# Autodesk Inventor assembly: Leg V4
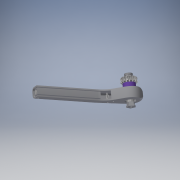
[picture p0: Inventor's stored thumbnail of the model, 180x180]
Saved by Autodesk Inventor 2019.1 (Build 231200000, 200)
## iProperties
Created: 2018-11-28
Part Number: Leg V4
Material: Generisch
Document SubType Name: Assembly
Designer: JochenAlt
Author: JochenAlt
## Documents named in this file (11)
- D:\Projects\Ondine\CAD\Leg\Leg V4.iam
- D:\Projects\Ondine\CAD\Leg\Leg V4.ipt
- D:\Projects\Ondine\CAD\Leg\Leg Inner V4.ipt
- D:\Projects\Ondine\CAD\Leg\LegInnerGear\Synchrone Riemenscheibe21.ipt
- D:\Projects\Ondine\CAD\Leg\LegInnerGear\Synchrone Riemenscheibe11.ipt
- D:\Projects\Ondine\CAD\Leg\LegInnerGear\Flache Riemenscheibe11.ipt
- D:\Projects\Ondine\CAD\Leg\LegInnerGear\Synchrone Riemenscheibe31.ipt
- D:\Projects\Ondine\CAD\Leg\Schnecke\Schneckenrad1.ipt
- D:\Projects\Ondine\CAD\Leg\LegInnerGear\gearNotch.ipt
- D:\Projects\Ondine\CAD\Bearings\W 627_7-2ZS.iam
- D:\Projects\Ondine\CAD\Bearings\W 61700 X-2RS1.iam
## Components (10 placed, 9 different names)
1. Leg:1 — Passend:7, Passend:8, Passend:23, Passend:24, Passend:26, Passend:27, Passend:28, Passend:29, Passend:30, Winkel:3, Passend:40, Passend:42
2. Leg:2 — Passend:41, Passend:42
3. Synchrone Riemenscheibe2:1 — Passend:26, Passend:27, Drehung:2, Passend:41
4. Synchrone Riemenscheibe1:1 — Passend:7, Passend:8, Passend:30
5. Flache Riemenscheibe1:1 — Passend:28, Passend:29
6. Synchrone Riemenscheibe3:1 — Winkel:2, Passend:21, Passend:23, Passend:24, Passend:25, Passend:33, Passend:34
7. LegGearWormPinion:1 — Passend:37, Passend:38, Winkel:3, Passend:39, Passend:40
8. gearNotch:1 — Winkel:2, Passend:21, Passend:25, Drehung:2
9. W 627_7-2ZS:1 [sub-assembly] — Passend:37, Passend:38
10. W 61700 X-2RS1:1 [sub-assembly] — Passend:33, Passend:34, Passend:39
## Relationships (22: Mate 19, Angle 2, RelateRotation 1)
- Passend:7 [Mate]: Leg:1 ↔ Synchrone Riemenscheibe1:1
- Passend:8 [Mate]: Leg:1 ↔ Synchrone Riemenscheibe1:1
- Winkel:2 [Angle] (180 deg): Synchrone Riemenscheibe3:1 ↔ gearNotch:1
- Passend:21 [Mate]: Synchrone Riemenscheibe3:1 ↔ gearNotch:1
- Passend:23 [Mate]: Leg:1 ↔ Synchrone Riemenscheibe3:1
- Passend:24 [Mate]: Leg:1 ↔ Synchrone Riemenscheibe3:1
- Passend:25 [Mate]: Synchrone Riemenscheibe3:1 ↔ gearNotch:1
- Passend:26 [Mate]: Leg:1 ↔ Synchrone Riemenscheibe2:1
- Passend:27 [Mate]: Leg:1 ↔ Synchrone Riemenscheibe2:1
- Passend:28 [Mate]: Leg:1 ↔ Flache Riemenscheibe1:1
- Passend:29 [Mate]: Leg:1 ↔ Flache Riemenscheibe1:1
- Passend:30 [Mate]: Leg:1 ↔ Synchrone Riemenscheibe1:1
- Passend:33 [Mate]: Synchrone Riemenscheibe3:1 ↔ W 61700 X-2RS1:1
- Passend:34 [Mate]: Synchrone Riemenscheibe3:1 ↔ W 61700 X-2RS1:1
- Drehung:2 [RelateRotation] (1 ul): Synchrone Riemenscheibe2:1 ↔ gearNotch:1
- Passend:37 [Mate]: LegGearWormPinion:1 ↔ W 627_7-2ZS:1
- Passend:38 [Mate]: LegGearWormPinion:1 ↔ W 627_7-2ZS:1
- Winkel:3 [Angle] (180 deg): Leg:1 ↔ LegGearWormPinion:1
- Passend:39 [Mate]: LegGearWormPinion:1 ↔ W 61700 X-2RS1:1
- Passend:40 [Mate]: Leg:1 ↔ LegGearWormPinion:1
- Passend:41 [Mate]: Leg:2 ↔ Synchrone Riemenscheibe2:1
- Passend:42 [Mate] (1 mm): Leg:1 ↔ Leg:2
